# Autodesk Inventor assembly: PG600 SKU 0 3D Model
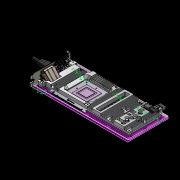
[picture p0: Inventor's stored thumbnail of the model, 180x180]
Saved by Autodesk Inventor 2018 (Build 220112000, 112)
## iProperties
Created: 2016-09-10
Part Number: PG600 SKU 0 3D Model
Material: 一般
Document SubType Name: Assembly
Designer: gisen
Sending System: SolidWorks 2016
Last Author: YDX
Last Saved: 2016-09-25
Author: gisen
## Documents named in this file (100)
- C:\Users\gisen\Documents\CAD\inventor\git\eatx_case\eatx_full\resources\nvidia-gtx980\Solidworks File (better version)\PG600 SKU 0 3D Model.iam
- C:\Users\gisen\Documents\CAD\inventor\git\eatx_case\eatx_full\resources\nvidia-gtx980\Solidworks File (better version)\142-1G600-1000-A05.ipt
- C:\Users\gisen\Documents\CAD\inventor\git\eatx_case\eatx_full\resources\nvidia-gtx980\Solidworks File (better version)\085-0009-000_1.ipt
- C:\Users\gisen\Documents\CAD\inventor\git\eatx_case\eatx_full\resources\nvidia-gtx980\Solidworks File (better version)\075-0186-000_1.ipt
- C:\Users\gisen\Documents\CAD\inventor\git\eatx_case\eatx_full\resources\nvidia-gtx980\Solidworks File (better version)\092-0023-000_1.ipt
- C:\Users\gisen\Documents\CAD\inventor\git\eatx_case\eatx_full\resources\nvidia-gtx980\Solidworks File (better version)\041-0139-000_1.ipt
- C:\Users\gisen\Documents\CAD\inventor\git\eatx_case\eatx_full\resources\nvidia-gtx980\Solidworks File (better version)\CAP_SMD_066X066_B_6000_GREY.ipt
- C:\Users\gisen\Documents\CAD\inventor\git\eatx_case\eatx_full\resources\nvidia-gtx980\Solidworks File (better version)\080-1128-000_3.ipt
- C:\Users\gisen\Documents\CAD\inventor\git\eatx_case\eatx_full\resources\nvidia-gtx980\Solidworks File (better version)\032-0286-000_1.ipt
- C:\Users\gisen\Documents\CAD\inventor\git\eatx_case\eatx_full\resources\nvidia-gtx980\Solidworks File (better version)\065-0573-000_3.ipt
- C:\Users\gisen\Documents\CAD\inventor\git\eatx_case\eatx_full\resources\nvidia-gtx980\Solidworks File (better version)\195-2659-000_1.ipt
- C:\Users\gisen\Documents\CAD\inventor\git\eatx_case\eatx_full\resources\nvidia-gtx980\Solidworks File (better version)\039-0122-000_1.ipt
- C:\Users\gisen\Documents\CAD\inventor\git\eatx_case\eatx_full\resources\nvidia-gtx980\Solidworks File (better version)\039-0127-000_1.ipt
- C:\Users\gisen\Documents\CAD\inventor\git\eatx_case\eatx_full\resources\nvidia-gtx980\Solidworks File (better version)\039-0123-000_1.ipt
- C:\Users\gisen\Documents\CAD\inventor\git\eatx_case\eatx_full\resources\nvidia-gtx980\Solidworks File (better version)\039-0183-000_1.ipt
- C:\Users\gisen\Documents\CAD\inventor\git\eatx_case\eatx_full\resources\nvidia-gtx980\Solidworks File (better version)\195-1593-000_1.ipt
- C:\Users\gisen\Documents\CAD\inventor\git\eatx_case\eatx_full\resources\nvidia-gtx980\Solidworks File (better version)\039-0149-000_1.ipt
- C:\Users\gisen\Documents\CAD\inventor\git\eatx_case\eatx_full\resources\nvidia-gtx980\Solidworks File (better version)\039-0128-000_1.ipt
- C:\Users\gisen\Documents\CAD\inventor\git\eatx_case\eatx_full\resources\nvidia-gtx980\Solidworks File (better version)\039-0186-000_1.ipt
- C:\Users\gisen\Documents\CAD\inventor\git\eatx_case\eatx_full\resources\nvidia-gtx980\Solidworks File (better version)\130-0445-000_2.ipt
- C:\Users\gisen\Documents\CAD\inventor\git\eatx_case\eatx_full\resources\nvidia-gtx980\Solidworks File (better version)\115-1357-000_2.ipt
- C:\Users\gisen\Documents\CAD\inventor\git\eatx_case\eatx_full\resources\nvidia-gtx980\Solidworks File (better version)\065-0301-000_1.ipt
- C:\Users\gisen\Documents\CAD\inventor\git\eatx_case\eatx_full\resources\nvidia-gtx980\Solidworks File (better version)\041-0188-000_1.ipt
- C:\Users\gisen\Documents\CAD\inventor\git\eatx_case\eatx_full\resources\nvidia-gtx980\Solidworks File (better version)\041-0190-000_2.ipt
- C:\Users\gisen\Documents\CAD\inventor\git\eatx_case\eatx_full\resources\nvidia-gtx980\Solidworks File (better version)\041-0085-000_2.ipt
- C:\Users\gisen\Documents\CAD\inventor\git\eatx_case\eatx_full\resources\nvidia-gtx980\Solidworks File (better version)\032-0070-000_1.ipt
- C:\Users\gisen\Documents\CAD\inventor\git\eatx_case\eatx_full\resources\nvidia-gtx980\Solidworks File (better version)\041-0196-000_1.ipt
- C:\Users\gisen\Documents\CAD\inventor\git\eatx_case\eatx_full\resources\nvidia-gtx980\Solidworks File (better version)\032-0299-000_1.ipt
- C:\Users\gisen\Documents\CAD\inventor\git\eatx_case\eatx_full\resources\nvidia-gtx980\Solidworks File (better version)\100-0028-000_1.ipt
- C:\Users\gisen\Documents\CAD\inventor\git\eatx_case\eatx_full\resources\nvidia-gtx980\Solidworks File (better version)\315-0756-000_1.ipt
- C:\Users\gisen\Documents\CAD\inventor\git\eatx_case\eatx_full\resources\nvidia-gtx980\Solidworks File (better version)\115-0121-000_1.ipt
- C:\Users\gisen\Documents\CAD\inventor\git\eatx_case\eatx_full\resources\nvidia-gtx980\Solidworks File (better version)\115-0398-000_1.ipt
- C:\Users\gisen\Documents\CAD\inventor\git\eatx_case\eatx_full\resources\nvidia-gtx980\Solidworks File (better version)\300-0766-000_1.ipt
- C:\Users\gisen\Documents\CAD\inventor\git\eatx_case\eatx_full\resources\nvidia-gtx980\Solidworks File (better version)\316-0134-000_3.ipt
- C:\Users\gisen\Documents\CAD\inventor\git\eatx_case\eatx_full\resources\nvidia-gtx980\Solidworks File (better version)\315-0829-000_4.ipt
- C:\Users\gisen\Documents\CAD\inventor\git\eatx_case\eatx_full\resources\nvidia-gtx980\Solidworks File (better version)\305-0092-000_1.ipt
- C:\Users\gisen\Documents\CAD\inventor\git\eatx_case\eatx_full\resources\nvidia-gtx980\Solidworks File (better version)\115-1286-000_2.ipt
- C:\Users\gisen\Documents\CAD\inventor\git\eatx_case\eatx_full\resources\nvidia-gtx980\Solidworks File (better version)\161-0163-100_1.ipt
- C:\Users\gisen\Documents\CAD\inventor\git\eatx_case\eatx_full\resources\nvidia-gtx980\Solidworks File (better version)\131-0786-000_1.ipt
- C:\Users\gisen\Documents\CAD\inventor\git\eatx_case\eatx_full\resources\nvidia-gtx980\Solidworks File (better version)\115-0732-000_1.ipt
- C:\Users\gisen\Documents\CAD\inventor\git\eatx_case\eatx_full\resources\nvidia-gtx980\Solidworks File (better version)\115-0967-000_1.ipt
- C:\Users\gisen\Documents\CAD\inventor\git\eatx_case\eatx_full\resources\nvidia-gtx980\Solidworks File (better version)\300-0250-000_1.ipt
- C:\Users\gisen\Documents\CAD\inventor\git\eatx_case\eatx_full\resources\nvidia-gtx980\Solidworks File (better version)\300-0787-000_1.ipt
- C:\Users\gisen\Documents\CAD\inventor\git\eatx_case\eatx_full\resources\nvidia-gtx980\Solidworks File (better version)\131-0213-000_2.ipt
- C:\Users\gisen\Documents\CAD\inventor\git\eatx_case\eatx_full\resources\nvidia-gtx980\Solidworks File (better version)\215-0139-000_2.ipt
- C:\Users\gisen\Documents\CAD\inventor\git\eatx_case\eatx_full\resources\nvidia-gtx980\Solidworks File (better version)\080-0424-000_1.ipt
- C:\Users\gisen\Documents\CAD\inventor\git\eatx_case\eatx_full\resources\nvidia-gtx980\Solidworks File (better version)\300-0667-000_1.ipt
- C:\Users\gisen\Documents\CAD\inventor\git\eatx_case\eatx_full\resources\nvidia-gtx980\Solidworks File (better version)\065-0415-000_2.ipt
- C:\Users\gisen\Documents\CAD\inventor\git\eatx_case\eatx_full\resources\nvidia-gtx980\Solidworks File (better version)\131-0560-000_2.ipt
- C:\Users\gisen\Documents\CAD\inventor\git\eatx_case\eatx_full\resources\nvidia-gtx980\Solidworks File (better version)\131-0397-000_2.ipt
- C:\Users\gisen\Documents\CAD\inventor\git\eatx_case\eatx_full\resources\nvidia-gtx980\Solidworks File (better version)\131-0134-000_3.ipt
- C:\Users\gisen\Documents\CAD\inventor\git\eatx_case\eatx_full\resources\nvidia-gtx980\Solidworks File (better version)\131-0257-000_1.ipt
- C:\Users\gisen\Documents\CAD\inventor\git\eatx_case\eatx_full\resources\nvidia-gtx980\Solidworks File (better version)\090-0091-000_2.ipt
- C:\Users\gisen\Documents\CAD\inventor\git\eatx_case\eatx_full\resources\nvidia-gtx980\Solidworks File (better version)\131-0246-000_2.ipt
- C:\Users\gisen\Documents\CAD\inventor\git\eatx_case\eatx_full\resources\nvidia-gtx980\Solidworks File (better version)\115-1066-000_2.ipt
- C:\Users\gisen\Documents\CAD\inventor\git\eatx_case\eatx_full\resources\nvidia-gtx980\Solidworks File (better version)\039-0125-000_1.ipt
- C:\Users\gisen\Documents\CAD\inventor\git\eatx_case\eatx_full\resources\nvidia-gtx980\Solidworks File (better version)\039-0135-000_1.ipt
- C:\Users\gisen\Documents\CAD\inventor\git\eatx_case\eatx_full\resources\nvidia-gtx980\Solidworks File (better version)\039-0037-000_1.ipt
- C:\Users\gisen\Documents\CAD\inventor\git\eatx_case\eatx_full\resources\nvidia-gtx980\Solidworks File (better version)\036-0043-000_1.ipt
- C:\Users\gisen\Documents\CAD\inventor\git\eatx_case\eatx_full\resources\nvidia-gtx980\Solidworks File (better version)\039-0227-000_1.ipt
- C:\Users\gisen\Documents\CAD\inventor\git\eatx_case\eatx_full\resources\nvidia-gtx980\Solidworks File (better version)\300-0602-000_1.ipt
- C:\Users\gisen\Documents\CAD\inventor\git\eatx_case\eatx_full\resources\nvidia-gtx980\Solidworks File (better version)\300-0484-000_2.ipt
- C:\Users\gisen\Documents\CAD\inventor\git\eatx_case\eatx_full\resources\nvidia-gtx980\Solidworks File (better version)\091-0002-000_1.ipt
- C:\Users\gisen\Documents\CAD\inventor\git\eatx_case\eatx_full\resources\nvidia-gtx980\Solidworks File (better version)\305-0005-000_1.ipt
- C:\Users\gisen\Documents\CAD\inventor\git\eatx_case\eatx_full\resources\nvidia-gtx980\Solidworks File (better version)\300-0675-000_1.ipt
- C:\Users\gisen\Documents\CAD\inventor\git\eatx_case\eatx_full\resources\nvidia-gtx980\Solidworks File (better version)\091-0016-000_1.ipt
- C:\Users\gisen\Documents\CAD\inventor\git\eatx_case\eatx_full\resources\nvidia-gtx980\Solidworks File (better version)\090-0085-000_1.ipt
- C:\Users\gisen\Documents\CAD\inventor\git\eatx_case\eatx_full\resources\nvidia-gtx980\Solidworks File (better version)\GM200-INT624126-A1_2.ipt
- C:\Users\gisen\Documents\CAD\inventor\git\eatx_case\eatx_full\resources\nvidia-gtx980\Solidworks File (better version)\115-0569-000_2.ipt
- C:\Users\gisen\Documents\CAD\inventor\git\eatx_case\eatx_full\resources\nvidia-gtx980\Solidworks File (better version)\170-0165-000_1.ipt
- C:\Users\gisen\Documents\CAD\inventor\git\eatx_case\eatx_full\resources\nvidia-gtx980\Solidworks File (better version)\315-0378-000_2.ipt
- C:\Users\gisen\Documents\CAD\inventor\git\eatx_case\eatx_full\resources\nvidia-gtx980\Solidworks File (better version)\316-0349-000_2.ipt
- C:\Users\gisen\Documents\CAD\inventor\git\eatx_case\eatx_full\resources\nvidia-gtx980\Solidworks File (better version)\315-0861-000_1.ipt
- C:\Users\gisen\Documents\CAD\inventor\git\eatx_case\eatx_full\resources\nvidia-gtx980\Solidworks File (better version)\065-0416-000_1.ipt
- C:\Users\gisen\Documents\CAD\inventor\git\eatx_case\eatx_full\resources\nvidia-gtx980\Solidworks File (better version)\130-0209-000_1.ipt
- C:\Users\gisen\Documents\CAD\inventor\git\eatx_case\eatx_full\resources\nvidia-gtx980\Solidworks File (better version)\130-0008-000_1.ipt
- C:\Users\gisen\Documents\CAD\inventor\git\eatx_case\eatx_full\resources\nvidia-gtx980\Solidworks File (better version)\100-0012-000_1.ipt
- C:\Users\gisen\Documents\CAD\inventor\git\eatx_case\eatx_full\resources\nvidia-gtx980\Solidworks File (better version)\100-0026-000_1.ipt
- C:\Users\gisen\Documents\CAD\inventor\git\eatx_case\eatx_full\resources\nvidia-gtx980\Solidworks File (better version)\100-0111-000_1.ipt
- C:\Users\gisen\Documents\CAD\inventor\git\eatx_case\eatx_full\resources\nvidia-gtx980\Solidworks File (better version)\1005_0600_GREY.ipt
- C:\Users\gisen\Documents\CAD\inventor\git\eatx_case\eatx_full\resources\nvidia-gtx980\Solidworks File (better version)\1005_BGA_0600_GREY.ipt
- C:\Users\gisen\Documents\CAD\inventor\git\eatx_case\eatx_full\resources\nvidia-gtx980\Solidworks File (better version)\215-0201-000_1.ipt
- C:\Users\gisen\Documents\CAD\inventor\git\eatx_case\eatx_full\resources\nvidia-gtx980\Solidworks File (better version)\195-1635-000_1.ipt
- C:\Users\gisen\Documents\CAD\inventor\git\eatx_case\eatx_full\resources\nvidia-gtx980\Solidworks File (better version)\195-1589-000_1.ipt
- C:\Users\gisen\Documents\CAD\inventor\git\eatx_case\eatx_full\resources\nvidia-gtx980\Solidworks File (better version)\039-0189-000_1.ipt
- C:\Users\gisen\Documents\CAD\inventor\git\eatx_case\eatx_full\resources\nvidia-gtx980\Solidworks File (better version)\106-0037-000_2.ipt
- C:\Users\gisen\Documents\CAD\inventor\git\eatx_case\eatx_full\resources\nvidia-gtx980\Solidworks File (better version)\115-0596-000_1.ipt
- C:\Users\gisen\Documents\CAD\inventor\git\eatx_case\eatx_full\resources\nvidia-gtx980\Solidworks File (better version)\115-1426-000_1.ipt
- C:\Users\gisen\Documents\CAD\inventor\git\eatx_case\eatx_full\resources\nvidia-gtx980\Solidworks File (better version)\131-0307-000_2.ipt
- C:\Users\gisen\Documents\CAD\inventor\git\eatx_case\eatx_full\resources\nvidia-gtx980\Solidworks File (better version)\131-0707-000_1.ipt
- C:\Users\gisen\Documents\CAD\inventor\git\eatx_case\eatx_full\resources\nvidia-gtx980\Solidworks File (better version)\131-0669-000_1.ipt
- C:\Users\gisen\Documents\CAD\inventor\git\eatx_case\eatx_full\resources\nvidia-gtx980\Solidworks File (better version)\131-0622-000_1.ipt
- C:\Users\gisen\Documents\CAD\inventor\git\eatx_case\eatx_full\resources\nvidia-gtx980\Solidworks File (better version)\074-0098-000_2.ipt
- C:\Users\gisen\Documents\CAD\inventor\git\eatx_case\eatx_full\resources\nvidia-gtx980\Solidworks File (better version)\065-00044-0000-000_1.ipt
- C:\Users\gisen\Documents\CAD\inventor\git\eatx_case\eatx_full\resources\nvidia-gtx980\Solidworks File (better version)\244-12203-1000-A01_ASM.iam
- C:\Users\gisen\Documents\CAD\inventor\git\eatx_case\eatx_full\resources\nvidia-gtx980\Solidworks File (better version)\682-1G600-0000-000_ASM.iam
- C:\Users\gisen\Documents\CAD\inventor\git\eatx_case\eatx_full\resources\nvidia-gtx980\Solidworks File (better version)\155-0166-000-MODEL.ipt
- C:\Users\gisen\Documents\CAD\inventor\git\eatx_case\eatx_full\resources\nvidia-gtx980\Solidworks File (better version)\065-0581-000_2 - OK.ipt
- C:\Users\gisen\Documents\CAD\inventor\git\eatx_case\eatx_full\resources\nvidia-gtx980\inventor\Part205.ipt
- C:\Users\gisen\Documents\CAD\inventor\git\eatx_case\eatx_full\resources\nvidia-gtx980\inventor\Part205_MIR.ipt
## Components (537 placed, 99 different names)
1. 142-1G600-1000-A05:1 — フラッシュ:1, フラッシュ:2
2. 085-0009-000_1:1
3. 075-0186-000_1:1
4. 092-0023-000_1:1
5. 041-0139-000_1:1
6. 041-0139-000_1:2
7. CAP_SMD_066X066_B_6000_GREY:1
8. CAP_SMD_066X066_B_6000_GREY:2
9. CAP_SMD_066X066_B_6000_GREY:3
10. CAP_SMD_066X066_B_6000_GREY:4
11. CAP_SMD_066X066_B_6000_GREY:5
12. CAP_SMD_066X066_B_6000_GREY:6
13. 080-1128-000_3:1
14. 080-1128-000_3:2
15. 080-1128-000_3:3
16. 032-0286-000_1:1
17. 032-0286-000_1:2
18. 032-0286-000_1:3
19. 032-0286-000_1:4
20. 032-0286-000_1:5
21. 032-0286-000_1:6
22. 065-0573-000_3:1
23. 195-2659-000_1:1
24. 195-2659-000_1:2
25. 039-0122-000_1:1
26. 039-0122-000_1:2
27. 039-0127-000_1:1
28. 039-0123-000_1:1
29. 039-0123-000_1:2
30. 039-0123-000_1:3
31. 039-0123-000_1:4
32. 039-0123-000_1:5
33. 039-0123-000_1:6
34. 039-0123-000_1:7
35. 039-0123-000_1:8
36. 195-2659-000_1:3
37. 195-2659-000_1:4
38. 039-0122-000_1:3
39. 039-0183-000_1:1
40. 039-0123-000_1:9
41. 039-0123-000_1:10
42. 039-0123-000_1:11
43. 039-0123-000_1:12
44. 195-1593-000_1:1
45. 195-1593-000_1:2
46. 039-0123-000_1:13
47. 039-0123-000_1:14
48. 039-0123-000_1:15
49. 039-0123-000_1:16
50. 039-0123-000_1:17
51. 039-0123-000_1:18
52. 039-0123-000_1:19
53. 039-0123-000_1:20
54. 039-0123-000_1:21
55. 039-0149-000_1:1
56. 039-0122-000_1:4
57. 039-0122-000_1:5
58. 039-0123-000_1:22
59. 039-0123-000_1:23
60. 039-0122-000_1:6
61. 039-0127-000_1:2
62. 039-0122-000_1:7
63. 039-0123-000_1:24
64. 039-0123-000_1:25
65. 039-0123-000_1:26
66. 039-0123-000_1:27
67. 039-0127-000_1:3
68. 039-0127-000_1:4
69. 039-0123-000_1:28
70. 039-0127-000_1:5
71. 039-0127-000_1:6
72. 039-0127-000_1:7
73. 039-0127-000_1:8
74. 039-0127-000_1:9
75. 039-0127-000_1:10
76. 039-0127-000_1:11
77. 039-0127-000_1:12
78. 039-0127-000_1:13
79. 039-0127-000_1:14
80. 039-0123-000_1:29
81. 039-0123-000_1:30
82. 039-0123-000_1:31
83. 039-0123-000_1:32
84. 039-0123-000_1:33
85. 039-0183-000_1:2
86. 195-2659-000_1:5
87. 039-0123-000_1:34
88. 039-0123-000_1:35
89. 039-0123-000_1:36
90. 039-0123-000_1:37
91. 039-0123-000_1:38
92. 039-0123-000_1:39
93. 039-0123-000_1:40
94. 039-0123-000_1:41
95. 039-0123-000_1:42
96. 039-0123-000_1:43
97. 039-0123-000_1:44
98. 039-0123-000_1:45
99. 039-0123-000_1:46
100. 039-0123-000_1:47
101. 039-0123-000_1:48
102. 039-0122-000_1:8
103. 039-0123-000_1:49
104. 039-0123-000_1:50
105. 039-0122-000_1:9
106. 039-0123-000_1:51
107. 039-0123-000_1:52
108. 039-0122-000_1:10
109. 039-0183-000_1:3
110. 039-0183-000_1:4
111. 039-0183-000_1:5
112. 039-0183-000_1:6
113. 039-0183-000_1:7
114. 039-0183-000_1:8
115. 039-0183-000_1:9
116. 039-0183-000_1:10
117. 039-0183-000_1:11
118. 039-0183-000_1:12
119. 039-0183-000_1:13
120. 039-0183-000_1:14
121. 039-0183-000_1:15
122. 039-0183-000_1:16
123. 039-0183-000_1:17
124. 039-0183-000_1:18
125. 039-0183-000_1:19
126. 039-0183-000_1:20
127. 039-0183-000_1:21
128. 039-0183-000_1:22
129. 039-0123-000_1:53
130. 039-0128-000_1:1
131. 039-0123-000_1:54
132. 039-0186-000_1:1
133. 039-0186-000_1:2
134. 195-2659-000_1:6
135. 195-2659-000_1:7
136. 195-2659-000_1:8
137. 195-2659-000_1:9
138. 130-0445-000_2:1
139. 130-0445-000_2:2
140. 115-1357-000_2:1
141. 115-1357-000_2:2
142. 065-0301-000_1:1
143. 041-0188-000_1:1
144. 041-0188-000_1:2
145. 041-0190-000_2:1
146. 041-0085-000_2:1
147. 041-0085-000_2:2
148. 032-0070-000_1:1
149. 032-0070-000_1:2
150. 032-0070-000_1:3
151. 032-0070-000_1:4
152. 032-0070-000_1:5
153. 032-0070-000_1:6
154. 032-0070-000_1:7
155. 032-0070-000_1:8
156. 041-0196-000_1:1
157. 032-0070-000_1:9
158. 041-0085-000_2:3
159. 041-0085-000_2:4
160. 041-0085-000_2:5
161. 041-0085-000_2:6
162. 041-0196-000_1:2
163. 041-0085-000_2:7
164. 041-0085-000_2:8
165. 041-0085-000_2:9
166. 041-0196-000_1:3
167. 041-0196-000_1:4
168. 041-0196-000_1:5
169. 041-0196-000_1:6
170. 041-0196-000_1:7
171. 041-0085-000_2:10
172. 041-0085-000_2:11
173. 041-0085-000_2:12
174. 041-0085-000_2:13
175. 041-0085-000_2:14
176. 041-0085-000_2:15
177. 041-0190-000_2:2
178. 041-0085-000_2:16
179. 041-0190-000_2:3
180. 032-0299-000_1:1
181. 032-0299-000_1:2
182. 032-0299-000_1:3
183. 100-0028-000_1:1
184. 100-0028-000_1:2
185. 100-0028-000_1:3
186. 315-0756-000_1:1
187. 115-0121-000_1:1
188. 115-0398-000_1:1
189. 300-0766-000_1:1
190. 316-0134-000_3:1
191. 315-0829-000_4:1
192. 305-0092-000_1:1
193. 115-1286-000_2:1
194. 161-0163-100_1:1
195. 161-0163-100_1:2
196. 161-0163-100_1:3
197. 161-0163-100_1:4
198. 161-0163-100_1:5
199. 161-0163-100_1:6
200. 161-0163-100_1:7
201. 161-0163-100_1:8
202. 161-0163-100_1:9
203. 161-0163-100_1:10
204. 161-0163-100_1:11
205. 161-0163-100_1:12
206. 161-0163-100_1:13
207. 161-0163-100_1:14
208. 161-0163-100_1:15
209. 161-0163-100_1:16
210. 161-0163-100_1:17
211. 161-0163-100_1:18
212. 161-0163-100_1:19
213. 161-0163-100_1:20
214. 161-0163-100_1:21
215. 161-0163-100_1:22
216. 161-0163-100_1:23
217. 161-0163-100_1:24
218. 131-0786-000_1:1
219. 131-0786-000_1:2
220. 115-0732-000_1:1
221. 115-0732-000_1:2
222. 115-0967-000_1:1
223. 115-0967-000_1:2
224. 300-0250-000_1:1
225. 300-0787-000_1:1
226. 300-0250-000_1:2
227. 300-0787-000_1:2
228. 131-0213-000_2:1
229. 215-0139-000_2:1
230. 215-0139-000_2:2
231. 215-0139-000_2:3
232. 080-0424-000_1:1
233. 300-0667-000_1:1
234. 300-0667-000_1:2
235. 300-0667-000_1:3
236. 065-0415-000_2:1
237. 131-0560-000_2:1
238. 131-0560-000_2:2
239. 131-0397-000_2:1
240. 131-0397-000_2:2
241. 131-0397-000_2:3
242. 131-0397-000_2:4
243. 131-0397-000_2:5
244. 131-0397-000_2:6
245. 131-0134-000_3:1
246. 131-0257-000_1:1
247. 131-0257-000_1:2
248. 090-0091-000_2:1
249. 131-0246-000_2:1
250. 115-1066-000_2:1
251. 039-0125-000_1:1
252. 039-0135-000_1:1
253. 039-0037-000_1:1
254. 039-0125-000_1:2
255. 039-0125-000_1:3
256. 039-0125-000_1:4
257. 039-0125-000_1:5
258. 039-0125-000_1:6
259. 039-0125-000_1:7
260. 039-0125-000_1:8
261. 039-0125-000_1:9
262. 039-0125-000_1:10
263. 039-0125-000_1:11
264. 039-0125-000_1:12
265. 039-0125-000_1:13
266. 039-0125-000_1:14
267. 039-0125-000_1:15
268. 039-0125-000_1:16
269. 039-0125-000_1:17
270. 039-0125-000_1:18
271. 039-0125-000_1:19
272. 039-0125-000_1:20
273. 039-0125-000_1:21
274. 039-0125-000_1:22
275. 039-0125-000_1:23
276. 039-0125-000_1:24
277. 039-0125-000_1:25
278. 039-0125-000_1:26
279. 039-0125-000_1:27
280. 039-0125-000_1:28
281. 039-0125-000_1:29
282. 039-0125-000_1:30
283. 039-0125-000_1:31
284. 039-0125-000_1:32
285. 039-0125-000_1:33
286. 039-0125-000_1:34
287. 039-0125-000_1:35
288. 039-0125-000_1:36
289. 039-0125-000_1:37
290. 039-0125-000_1:38
291. 039-0125-000_1:39
292. 039-0125-000_1:40
293. 039-0125-000_1:41
294. 039-0125-000_1:42
295. 039-0125-000_1:43
296. 039-0125-000_1:44
297. 036-0043-000_1:1
298. 036-0043-000_1:2
299. 036-0043-000_1:3
300. 036-0043-000_1:4
301. 039-0125-000_1:45
302. 039-0125-000_1:46
303. 039-0125-000_1:47
304. 036-0043-000_1:5
305. 036-0043-000_1:6
306. 036-0043-000_1:7
307. 036-0043-000_1:8
308. 036-0043-000_1:9
309. 039-0125-000_1:48
310. 039-0227-000_1:1
311. 039-0125-000_1:49
312. 039-0125-000_1:50
313. 039-0125-000_1:51
314. 039-0125-000_1:52
315. 039-0125-000_1:53
316. 039-0125-000_1:54
317. 039-0125-000_1:55
318. 036-0043-000_1:10
319. 036-0043-000_1:11
320. 036-0043-000_1:12
321. 039-0125-000_1:56
322. 039-0125-000_1:57
323. 039-0125-000_1:58
324. 039-0125-000_1:59
325. 039-0125-000_1:60
326. 039-0125-000_1:61
327. 039-0125-000_1:62
328. 039-0125-000_1:63
329. 039-0125-000_1:64
330. 039-0125-000_1:65
331. 039-0125-000_1:66
332. 039-0125-000_1:67
333. 039-0125-000_1:68
334. 039-0125-000_1:69
335. 039-0125-000_1:70
336. 036-0043-000_1:13
337. 039-0125-000_1:71
338. 039-0125-000_1:72
339. 039-0125-000_1:73
340. 039-0125-000_1:74
341. 039-0125-000_1:75
342. 039-0125-000_1:76
343. 039-0125-000_1:77
344. 039-0125-000_1:78
345. 039-0125-000_1:79
346. 039-0125-000_1:80
347. 039-0125-000_1:81
348. 039-0125-000_1:82
349. 039-0125-000_1:83
350. 039-0125-000_1:84
351. 039-0125-000_1:85
352. 039-0125-000_1:86
353. 039-0125-000_1:87
354. 039-0125-000_1:88
355. 300-0602-000_1:1
356. 300-0602-000_1:2
357. 300-0602-000_1:3
358. 300-0602-000_1:4
359. 300-0602-000_1:5
360. 300-0602-000_1:6
361. 300-0484-000_2:1
362. 091-0002-000_1:1
363. 091-0002-000_1:2
364. 091-0002-000_1:3
365. 300-0602-000_1:7
366. 300-0602-000_1:8
367. 300-0602-000_1:9
368. 300-0602-000_1:10
369. 091-0002-000_1:4
370. 300-0602-000_1:11
371. 305-0005-000_1:1
372. 305-0005-000_1:2
373. 305-0005-000_1:3
374. 305-0005-000_1:4
375. 305-0005-000_1:5
376. 300-0602-000_1:12
377. 300-0602-000_1:13
378. 300-0602-000_1:14
379. 300-0602-000_1:15
380. 300-0602-000_1:16
381. 300-0602-000_1:17
382. 300-0602-000_1:18
383. 300-0602-000_1:19
384. 300-0602-000_1:20
385. 300-0602-000_1:21
386. 300-0602-000_1:22
387. 300-0602-000_1:23
388. 300-0602-000_1:24
389. 300-0602-000_1:25
390. 305-0005-000_1:6
391. 305-0005-000_1:7
392. 300-0602-000_1:26
393. 305-0005-000_1:8
394. 300-0602-000_1:27
395. 300-0602-000_1:28
396. 300-0602-000_1:29
397. 300-0602-000_1:30
398. 300-0675-000_1:1
399. 091-0016-000_1:1
400. 305-0005-000_1:9
401. 300-0602-000_1:31
402. 300-0675-000_1:2
403. 305-0005-000_1:10
404. 091-0002-000_1:5
405. 091-0002-000_1:6
406. 300-0602-000_1:32
407. 300-0602-000_1:33
408. 300-0602-000_1:34
409. 300-0602-000_1:35
410. 300-0602-000_1:36
411. 305-0005-000_1:11
412. 305-0005-000_1:12
413. 305-0005-000_1:13
414. 305-0005-000_1:14
415. 300-0602-000_1:37
416. 300-0602-000_1:38
417. 091-0002-000_1:7
418. 091-0002-000_1:8
419. 305-0005-000_1:15
420. 091-0002-000_1:9
421. 090-0085-000_1:1
422. 305-0005-000_1:16
423. 300-0602-000_1:39
424. 305-0005-000_1:17
425. 300-0602-000_1:40
426. 300-0602-000_1:41
427. 305-0005-000_1:18
428. 300-0602-000_1:42
429. 300-0602-000_1:43
430. 300-0602-000_1:44
431. 300-0602-000_1:45
432. 305-0005-000_1:19
433. 305-0005-000_1:20
434. GM200-INT624126-A1_2:1
435. 115-0569-000_2:1
436. 170-0165-000_1:1
437. 115-0569-000_2:2
438. 315-0378-000_2:1
439. 316-0349-000_2:1
440. 316-0349-000_2:2
441. 316-0349-000_2:3
442. 316-0349-000_2:4
443. 316-0349-000_2:5
444. 316-0349-000_2:6
445. 316-0349-000_2:7
446. 316-0349-000_2:8
447. 315-0861-000_1:1
448. 065-0416-000_1:1
449. 130-0209-000_1:1
450. 130-0209-000_1:2
451. 130-0209-000_1:3
452. 130-0008-000_1:1
453. 100-0012-000_1:1
454. 100-0026-000_1:1
455. 130-0008-000_1:2
456. 100-0111-000_1:1
457. 100-0111-000_1:2
458. 100-0026-000_1:2
459. 100-0111-000_1:3
460. 1005_0600_GREY:1
461. 1005_0600_GREY:2
462. 1005_0600_GREY:3
463. 1005_0600_GREY:4
464. 1005_0600_GREY:5
465. 1005_0600_GREY:6
466. 1005_0600_GREY:7
467. 1005_BGA_0600_GREY:1
468. 1005_BGA_0600_GREY:2
469. 1005_BGA_0600_GREY:3
470. 1005_BGA_0600_GREY:4
471. 1005_BGA_0600_GREY:5
472. 1005_BGA_0600_GREY:6
473. 1005_BGA_0600_GREY:7
474. 1005_BGA_0600_GREY:8
475. 1005_BGA_0600_GREY:9
476. 1005_BGA_0600_GREY:10
477. 1005_BGA_0600_GREY:11
478. 1005_BGA_0600_GREY:12
479. 1005_BGA_0600_GREY:13
480. 1005_BGA_0600_GREY:14
481. 1005_BGA_0600_GREY:15
482. 1005_BGA_0600_GREY:16
483. 1005_BGA_0600_GREY:17
484. 1005_BGA_0600_GREY:18
485. 1005_BGA_0600_GREY:19
486. 1005_BGA_0600_GREY:20
487. 1005_BGA_0600_GREY:21
488. 1005_BGA_0600_GREY:22
489. 1005_BGA_0600_GREY:23
490. 1005_BGA_0600_GREY:24
491. 1005_BGA_0600_GREY:25
492. 1005_BGA_0600_GREY:26
493. 1005_BGA_0600_GREY:27
494. 215-0201-000_1:1
495. 195-1635-000_1:1
496. 195-1635-000_1:2
497. 195-1635-000_1:3
498. 195-1635-000_1:4
499. 195-1635-000_1:5
500. 195-1589-000_1:1
501. 195-1589-000_1:2
502. 039-0189-000_1:1
503. 039-0189-000_1:2
504. 195-1589-000_1:3
505. 195-1589-000_1:4
506. 195-1589-000_1:5
507. 195-1589-000_1:6
508. 195-1589-000_1:7
509. 195-1589-000_1:8
510. 106-0037-000_2:1
511. 039-0189-000_1:3
512. 039-0189-000_1:4
513. 039-0189-000_1:5
514. 115-0596-000_1:1
515. 115-0596-000_1:2
516. 115-0596-000_1:3
517. 115-0596-000_1:4
518. 115-0596-000_1:5
519. 115-0596-000_1:6
520. 115-0596-000_1:7
521. 115-1426-000_1:1
522. 115-1426-000_1:2
523. 115-0596-000_1:8
524. 131-0307-000_2:1
525. 131-0307-000_2:2
526. 131-0707-000_1:1
527. 131-0669-000_1:1
528. 131-0622-000_1:1
529. 074-0098-000_2:1
530. 065-00044-0000-000_1:1
531. 244-12203-1000-A01_ASM:1 [sub-assembly]
532. 682-1G600-0000-000_ASM:1 [sub-assembly]
533. 155-0166-000-MODEL:1
534. 155-0166-000-MODEL:2
535. 065-0581-000_2 - OK:1
536. Part205:1 — フラッシュ:3, フラッシュ:4, 対称度:1
537. Part205_MIR:1
## Relationships (5: Flush 4, Symmetry 1)
- フラッシュ:1 [Flush] (2.5 mm): 142-1G600-1000-A05:1
- フラッシュ:2 [Flush] (2.5 mm): 142-1G600-1000-A05:1
- フラッシュ:3 [Flush]: Part205:1
- フラッシュ:4 [Flush]: Part205:1
- 対称度:1 [Symmetry]: Part205:1
